# Autodesk Inventor assembly: prototype7
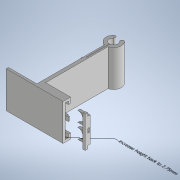
[picture p0: Inventor's stored thumbnail of the model, 180x180]
Saved by Autodesk Inventor 2022 (Build 260153000, 153)
## iProperties
Created: 2022-06-15
Part Number: prototype7
Document SubType Name: Assembly
Designer: tecware
Author: tecware
## Documents named in this file (3)
- C:\Users\tecware\Documents\git\calibrationKit\calibrationKit_v2\wand\prototype\prototype_8.iam
- C:\Users\tecware\Documents\git\calibrationKit\calibrationKit_v2\wand\prototype\prototype_8_1.ipt
- C:\Users\tecware\Documents\git\calibrationKit\calibrationKit_v2\wand\prototype\prototype_8_2.ipt
## Components (2 placed, 2 different names)
1. prototype_8_1:1 — Flush:1, Flush:2, Mate:1
2. prototype_8_2:1 — Flush:1, Flush:2, Mate:1
## Relationships (3: Flush 2, Mate 1)
- Flush:1: prototype_8_1:1 ↔ prototype_8_2:1
- Flush:2: prototype_8_1:1 ↔ prototype_8_2:1
- Mate:1 (0.2 mm): prototype_8_1:1 ↔ prototype_8_2:1
